# Autodesk Inventor assembly: ban baru assembly
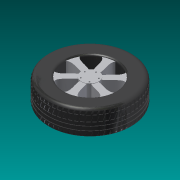
[picture p0: Inventor's stored thumbnail of the model, 180x180]
Saved by Autodesk Inventor 2014 SP2 (Build 180246200, 246)
## iProperties
Created: 2019-07-22
Part Number: ban baru assembly
Document SubType Name: Assembly
Designer: USER PC
Author: USER PC
## Documents named in this file (3)
- C:\Users\USER PC\Desktop\United Tractors\New folder\ban baru assembly.iam
- C:\Users\USER PC\Desktop\United Tractors\New folder\velg.ipt
- C:\Users\USER PC\Desktop\United Tractors\New folder\ban baru.ipt
## Components (2 placed, 2 different names)
1. velg:1 — Rotational:1, Rigid:1
2. ban baru:1 — Rotational:1, Rigid:1
## Relationships (2: RevoluteJoint 1, WeldJoint 1)
- Rotational:1 [RevoluteJoint] (-15 mm): velg:1 ↔ ban baru:1
- Rigid:1 [WeldJoint]: velg:1 ↔ ban baru:1
